# Autodesk Inventor assembly: CannonV2
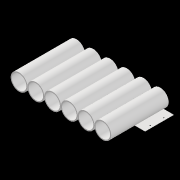
[picture p0: Inventor's stored thumbnail of the model, 180x180]
Saved by Autodesk Inventor 2022 (Build 260153000, 153)
## iProperties
Created: 2021-10-10
Part Number: CannonV2
Document SubType Name: Assembly
Designer: timmy
Author: timmy
## Documents named in this file (3)
- S:\Inventor\RoboCatz\T-Shirt\CannonV2.iam
- S:\Inventor\RoboCatz\T-Shirt\cannonplate.ipt
- S:\Inventor\RoboCatz\T-Shirt\3FT-SCH40-PVC.ipt
## Components (7 placed, 2 different names)
1. cannonplate:1 — Flush:1, Tangent:1, Tangent:4, Tangent:5, Tangent:6, Tangent:8, Tangent:9, Tangent:11
2. 3FT-SCH40-PVC:1 — Flush:1, Tangent:1, Tangent:2, Flush:2, Flush:3, Flush:4, Flush:5, Flush:11
3. 3FT-SCH40-PVC:2 — Tangent:2, Tangent:3, Tangent:4, Flush:5, Flush:10
4. 3FT-SCH40-PVC:3 — Tangent:3, Tangent:5, Tangent:7, Flush:4, Flush:9
5. 3FT-SCH40-PVC:4 — Tangent:6, Tangent:7, Tangent:8, Tangent:10, Flush:3, Flush:8
6. 3FT-SCH40-PVC:5 — Tangent:9, Tangent:10, Flush:2, Tangent:12, Flush:6, Flush:7
7. 3FT-SCH40-PVC:6 — Tangent:11, Tangent:12, Flush:6, Flush:7, Flush:8, Flush:9, Flush:10, Flush:11
## Relationships (23: Tangent 12, Flush 11)
- Flush:1: cannonplate:1 ↔ 3FT-SCH40-PVC:1
- Tangent:1: cannonplate:1 ↔ 3FT-SCH40-PVC:1
- Tangent:2: 3FT-SCH40-PVC:1 ↔ 3FT-SCH40-PVC:2
- Tangent:3: 3FT-SCH40-PVC:2 ↔ 3FT-SCH40-PVC:3
- Tangent:4: cannonplate:1 ↔ 3FT-SCH40-PVC:2
- Tangent:5: cannonplate:1 ↔ 3FT-SCH40-PVC:3
- Tangent:6: cannonplate:1 ↔ 3FT-SCH40-PVC:4
- Tangent:7: 3FT-SCH40-PVC:3 ↔ 3FT-SCH40-PVC:4
- Tangent:8: cannonplate:1 ↔ 3FT-SCH40-PVC:4
- Tangent:9: cannonplate:1 ↔ 3FT-SCH40-PVC:5
- Tangent:10: 3FT-SCH40-PVC:4 ↔ 3FT-SCH40-PVC:5
- Flush:2: 3FT-SCH40-PVC:1 ↔ 3FT-SCH40-PVC:5
- Flush:3: 3FT-SCH40-PVC:1 ↔ 3FT-SCH40-PVC:4
- Flush:4: 3FT-SCH40-PVC:1 ↔ 3FT-SCH40-PVC:3
- Flush:5: 3FT-SCH40-PVC:1 ↔ 3FT-SCH40-PVC:2
- Tangent:11: cannonplate:1 ↔ 3FT-SCH40-PVC:6
- Tangent:12: 3FT-SCH40-PVC:5 ↔ 3FT-SCH40-PVC:6
- Flush:6: 3FT-SCH40-PVC:5 ↔ 3FT-SCH40-PVC:6
- Flush:7: 3FT-SCH40-PVC:5 ↔ 3FT-SCH40-PVC:6
- Flush:8: 3FT-SCH40-PVC:4 ↔ 3FT-SCH40-PVC:6
- Flush:9: 3FT-SCH40-PVC:3 ↔ 3FT-SCH40-PVC:6
- Flush:10: 3FT-SCH40-PVC:2 ↔ 3FT-SCH40-PVC:6
- Flush:11: 3FT-SCH40-PVC:1 ↔ 3FT-SCH40-PVC:6
